# Autodesk Inventor assembly: robot assembly
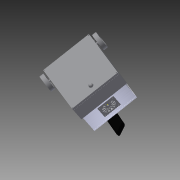
[picture p0: Inventor's stored thumbnail of the model, 180x180]
Saved by Autodesk Inventor 2015 (Build 190159000, 159)
## iProperties
Created: 2014-10-11
Part Number: robot assembly
Document SubType Name: Assembly
Designer: ericd_000
Author: ericd_000
## Documents named in this file (4)
- C:\Users\ericd_000\Dropbox\GitHub\initial_cad\eric_cad\robot assembly.iam
- C:\Users\ericd_000\Dropbox\GitHub\initial_cad\eric_cad\bottom box with container.iam
- C:\Users\ericd_000\Dropbox\GitHub\initial_cad\eric_cad\locomotion assembly.iam
- C:\Users\ericd_000\Dropbox\GitHub\initial_cad\eric_cad\perception module.iam
## Components (3 placed, 3 different names)
1. bottom box with container:1 [sub-assembly] — Mate:1, Flush:1, Mate:2, Mate:3, Flush:2
2. locomotion assembly:1 [sub-assembly] — Mate:1, Flush:1, Flush:2
3. perception module:1 [sub-assembly] — Mate:2, Mate:3
## Relationships (5: Mate 3, Flush 2)
- Mate:1: bottom box with container:1 ↔ locomotion assembly:1
- Flush:1 (10 mm): bottom box with container:1 ↔ locomotion assembly:1
- Mate:2: bottom box with container:1 ↔ perception module:1
- Mate:3: bottom box with container:1 ↔ perception module:1
- Flush:2 (10 mm): bottom box with container:1 ↔ locomotion assembly:1
